# Autodesk Inventor assembly: R-O v4
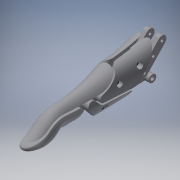
[picture p0: Inventor's stored thumbnail of the model, 180x180]
Saved by Autodesk Inventor 2018 (Build 220112000, 112)
## iProperties
Created: 2017-09-22
Part Number: R-O v4
Material: 一般
Document SubType Name: Assembly
Designer: sktom
Author: sktom
## Documents named in this file (9)
- D:\cloudstrage\NextCloud\Cad_mechanical\HACKberry_SizeM\3Dmodel\R\M-R-H\M-R-O\M-R-O.iam
- D:\cloudstrage\NextCloud\Cad_mechanical\HACKberry_SizeM\3Dmodel\R\M-R-H\M-R-O\M-R-O-other1.ipt
- D:\cloudstrage\NextCloud\Cad_mechanical\HACKberry_SizeM\3Dmodel\R\M-R-H\M-R-O\M-R-O-01.ipt
- D:\cloudstrage\NextCloud\Cad_mechanical\HACKberry_SizeM\3Dmodel\R\M-R-H\M-R-O\M-R-O-02.ipt
- D:\cloudstrage\NextCloud\Cad_mechanical\HACKberry_SizeM\3Dmodel\R\M-R-H\M-R-O\M-R-O-03.ipt
- D:\cloudstrage\NextCloud\Cad_mechanical\HACKberry_SizeM\3Dmodel\R\M-R-H\M-R-O\M-R-O-04.ipt
- D:\cloudstrage\NextCloud\Cad_mechanical\HACKberry_SizeM\3Dmodel\R\M-R-H\M-R-O\M-R-O-05.ipt
- D:\cloudstrage\NextCloud\Cad_mechanical\HACKberry_SizeM\3Dmodel\R\M-R-H\M-R-O\M1.7_L8.ipt
- D:\cloudstrage\NextCloud\Cad_mechanical\HACKberry_SizeM\3Dmodel\R\M-R-H\M-R-O\Shaft_phi2_L8.ipt
## Components (12 placed, 8 different names)
1. R-O-other1 v1:1 — 回転:1, 円柱状:1, 円柱状:2, 円柱状:3
2. R-O-01 v1:1 — 回転:1, 円柱状:1, 回転:5, リジッド:1, リジッド:2
3. R-O-02 v1:1 — 円柱状:2
4. R-O-03 v1:1 — 回転:3, 円柱状:3
5. R-O-04 v1:1 — 回転:3, 挿入:1, 挿入:2
6. R-O-05 v1:1 — 回転:5, 挿入:3, 挿入:4
7. M1.7_L8:1 — 挿入:1
8. M1.7_L8:2 — 挿入:2
9. M1.7_L8:3 — 挿入:3
10. M1.7_L8:4 — 挿入:4
11. Shaft_phi2_L8:1 — リジッド:1
12. Shaft_phi2_L8:2 — リジッド:2
## Relationships (12: Insert 4, RevoluteJoint 3, CylindricalJoint 3, WeldJoint 2)
- 回転:1 [RevoluteJoint]: R-O-other1 v1:1 ↔ R-O-01 v1:1
- 円柱状:1 [CylindricalJoint]: R-O-other1 v1:1 ↔ R-O-01 v1:1
- 回転:3 [RevoluteJoint]: R-O-03 v1:1 ↔ R-O-04 v1:1
- 回転:5 [RevoluteJoint] (-0.2 mm): R-O-01 v1:1 ↔ R-O-05 v1:1
- 円柱状:2 [CylindricalJoint]: R-O-other1 v1:1 ↔ R-O-02 v1:1
- 円柱状:3 [CylindricalJoint]: R-O-other1 v1:1 ↔ R-O-03 v1:1
- 挿入:1 [Insert]: R-O-04 v1:1 ↔ M1.7_L8:1
- 挿入:2 [Insert]: R-O-04 v1:1 ↔ M1.7_L8:2
- 挿入:3 [Insert]: R-O-05 v1:1 ↔ M1.7_L8:3
- 挿入:4 [Insert]: R-O-05 v1:1 ↔ M1.7_L8:4
- リジッド:1 [WeldJoint]: R-O-01 v1:1 ↔ Shaft_phi2_L8:1
- リジッド:2 [WeldJoint]: R-O-01 v1:1 ↔ Shaft_phi2_L8:2
